# Autodesk Inventor assembly: NDV-1000 Center 01
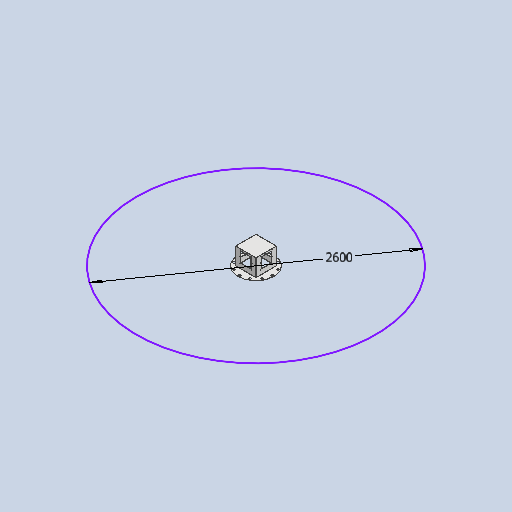
[picture p0: Inventor's stored thumbnail of the model, 512x512]
Saved by Autodesk Inventor 2026.2 (Build 302298000, 298)
## iProperties
Created: 2026-05-12
Part Number: NDV-1000 Center 01
Document SubType Name: Assembly
Designer: admin
Stock Number: Центр
Author: admin
## Documents named in this file (4)
- C:\Users\admin\Documents\Inventor\KND-DistribSystem\DRS_D1200\NDV-1000 Center 01.iam
- C:\Users\admin\Documents\Inventor\KND-DistribSystem\DRS_D1200\NDV-1103 Center flange 01.ipt
- C:\Users\admin\Documents\Inventor\KND-DistribSystem\DRS_D1200\NDV-1101 Center wall 01.ipt
- C:\Users\admin\Documents\Inventor\KND-DistribSystem\DRS_D1200\NDV-1102 Center cap 01.ipt
## Components (4 placed, 3 different names)
1. NDV-1103 Center flange 01:1 — Flush:8, Flush:7, Mate:3
2. NDV-1101 Center wall 01:1 — Flush:8, Flush:7, Mate:10, Rigid:22
3. NDV-1101 Center wall 01:2 — Mate:3, Rigid:22
4. NDV-1102 Center cap 01:1 — Mate:10
## Relationships (5: Flush 2, Mate 2, WeldJoint 1)
- Flush:8: NDV-1103 Center flange 01:1 ↔ NDV-1101 Center wall 01:1
- Flush:7: NDV-1103 Center flange 01:1 ↔ NDV-1101 Center wall 01:1
- Mate:10: NDV-1101 Center wall 01:1 ↔ NDV-1102 Center cap 01:1
- Mate:3: NDV-1103 Center flange 01:1 ↔ NDV-1101 Center wall 01:2
- Rigid:22 [WeldJoint]: NDV-1101 Center wall 01:1 ↔ NDV-1101 Center wall 01:2
